# Autodesk Inventor assembly: Hinge Assembly
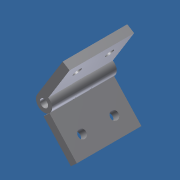
[picture p0: Inventor's stored thumbnail of the model, 180x180]
Saved by Autodesk Inventor 2012 (Build 160160000, 160)
## iProperties
Created: 2012-02-06
Part Number: Hinge Assembly
Document SubType Name: Assembly
Designer: Allison Garza
Author: Allison Garza
## Documents named in this file (3)
- C:\Users\Allison Garza\Documents\Rice Spring 2012\MRSL\Hinge Assembly.iam
- C:\Users\Allison Garza\Documents\Rice Spring 2012\MRSL\hinge two prong.ipt
- C:\Users\Allison Garza\Documents\Rice Spring 2012\MRSL\hinge one prong.ipt
## Components (2 placed, 2 different names)
1. hinge two prong:1 — Mate:1, Mate:2
2. hinge one prong:1 — Mate:1, Mate:2
## Relationships (2: Mate 2)
- Mate:1: hinge two prong:1 ↔ hinge one prong:1
- Mate:2: hinge two prong:1 ↔ hinge one prong:1
